# Autodesk Inventor assembly: printer
(part 3 of 3)
- [Mate]: 608RS:5 ↔ CSN 02 1702 B B 8,4:13
- [Mate]: 608RS:5 ↔ CSN 02 1702 B B 8,4:13
- [Mate]: 608RS:6 ↔ rope_pulley:8
- [Mate]: 608RS:6 ↔ rope_pulley:8
- [Mate]: rope_pulley:7 ↔ rope_pulley:8
- [Mate]: rope_pulley:7 ↔ rope_pulley:8
- [Mate]: 608RS:6 ↔ rope_pulley:7
- [Mate]: CSN 02 1702 B B 8,4:15 ↔ CSN 02 1702 B B 8,4:16
- [Mate]: CSN 02 1702 B B 8,4:15 ↔ CSN 02 1702 B B 8,4:16
- [Mate]: CSN 02 1702 B B 8,4:17 ↔ CSN 02 1702 B B 8,4:18
- [Mate]: CSN 02 1702 B B 8,4:17 ↔ CSN 02 1702 B B 8,4:18
- [Mate]: 608RS:6 ↔ CSN 02 1702 B B 8,4:15
- [Mate]: 608RS:6 ↔ CSN 02 1702 B B 8,4:15
- [Mate]: 608RS:6 ↔ CSN 02 1702 B B 8,4:17
- [Mate]: 608RS:6 ↔ CSN 02 1702 B B 8,4:17
- [Mate]: 608RS:7 ↔ rope_pulley:10
- [Mate]: 608RS:7 ↔ rope_pulley:10
- [Mate]: rope_pulley:9 ↔ rope_pulley:10
- [Mate]: rope_pulley:9 ↔ rope_pulley:10
- [Mate]: 608RS:7 ↔ rope_pulley:9
- [Mate]: CSN 02 1702 B B 8,4:19 ↔ CSN 02 1702 B B 8,4:20
- [Mate]: CSN 02 1702 B B 8,4:19 ↔ CSN 02 1702 B B 8,4:20
- [Mate]: CSN 02 1702 B B 8,4:21 ↔ CSN 02 1702 B B 8,4:22
- [Mate]: CSN 02 1702 B B 8,4:21 ↔ CSN 02 1702 B B 8,4:22
- [Mate]: 608RS:7 ↔ CSN 02 1702 B B 8,4:19
- [Mate]: 608RS:7 ↔ CSN 02 1702 B B 8,4:19
- [Mate]: 608RS:7 ↔ CSN 02 1702 B B 8,4:21
- [Mate]: 608RS:7 ↔ CSN 02 1702 B B 8,4:21
- Mate:607: rope_mount_b:1 ↔ CSN 02 1702 B B 8,4:14
- Mate:608: rope_mount_b:1 ↔ CSN 02 1702 B B 8,4:14
- Mate:609: rope_mount_b:1 ↔ CSN 02 1702 B B 8,4:18
- Mate:610: rope_mount_b:1 ↔ CSN 02 1702 B B 8,4:18
- Mate:611: rope_mount_b:2 ↔ CSN 02 1702 B B 8,4:22
- Mate:612: rope_mount_b:2 ↔ CSN 02 1702 B B 8,4:22
- Mate:613: rope_mount_b:2 ↔ CSN 02 1702 B B 8,4:10
- Mate:614: rope_mount_b:2 ↔ CSN 02 1702 B B 8,4:10
- Mate:615: rope_mount_b:2 ↔ CSN 02 1702 B B 8,4:30
- Mate:616: rope_mount_b:2 ↔ CSN 02 1702 B B 8,4:30
- Mate:617: rope_mount_b:2 ↔ CSN 02 1702 B B 8,4:29
- Mate:618: rope_mount_b:2 ↔ CSN 02 1702 B B 8,4:29
- Mate:619: rope_mount_a:1 ↔ CSN 02 1702 B B 8,4:28
- Mate:620: rope_mount_a:1 ↔ CSN 02 1702 B B 8,4:27
- Mate:621: rope_mount_b:1 ↔ CSN 02 1702 B B 8,4:26
- Mate:622: rope_mount_b:1 ↔ CSN 02 1702 B B 8,4:26
- Mate:623: rope_mount_b:1 ↔ CSN 02 1702 B B 8,4:25
- Mate:624: rope_mount_b:1 ↔ CSN 02 1702 B B 8,4:25
- Mate:625: rope_mount_a:2 ↔ CSN 02 1702 B B 8,4:24
- Mate:626: rope_mount_a:2 ↔ CSN 02 1702 B B 8,4:23
- Insert:133: CSN 02 1702 B B 8,4:30 ↔ ISO 4762 M8 x 40:5
- Insert:134: CSN 02 1702 B B 8,4:29 ↔ ISO 4762 M8 x 40:4
- Insert:135: CSN 02 1702 B B 8,4:26 ↔ ISO 4762 M8 x 40:3
- Insert:136: CSN 02 1702 B B 8,4:25 ↔ ISO 4762 M8 x 40:2
- Mate:627: CSN 02 1702 B B 8,4:24 ↔ ISO 4762 M8 x 40:5
- Mate:628: CSN 02 1702 B B 8,4:23 ↔ ISO 4762 M8 x 40:4
- Mate:629: CSN 02 1702 B B 8,4:28 ↔ ISO 4762 M8 x 40:3
- Mate:630: CSN 02 1702 B B 8,4:27 ↔ ISO 4762 M8 x 40:2
- Mate:631: CSN 02 1702 B B 8,4:23 ↔ DIN EN ISO 7040 M8:5
- Mate:632: ISO 4762 M8 x 40:4 ↔ DIN EN ISO 7040 M8:5
- Mate:633: CSN 02 1702 B B 8,4:24 ↔ DIN EN ISO 7040 M8:4
- Mate:634: ISO 4762 M8 x 40:5 ↔ DIN EN ISO 7040 M8:4
- Mate:635: CSN 02 1702 B B 8,4:27 ↔ DIN EN ISO 7040 M8:3
- Mate:636: ISO 4762 M8 x 40:2 ↔ DIN EN ISO 7040 M8:3
- Mate:637: CSN 02 1702 B B 8,4:28 ↔ DIN EN ISO 7040 M8:2
- Mate:638: ISO 4762 M8 x 40:3 ↔ DIN EN ISO 7040 M8:2
- Mate:639: frame:1 ↔ z_axis_top_brace:2
- Mate:640: frame:1 ↔ z_axis_top_brace:2
- Mate:641: z_axis_top:1 ↔ z_axis_top_brace:2
- Mate:642: frame:1 ↔ z_axis_top_brace:1
- Mate:643: z_axis_top:2 ↔ z_axis_top_brace:1
- Mate:644: frame:1 ↔ z_axis_top_brace:1
- Mate:645: z_axis_top:1 ↔ CSN 02 1702 B B 4,3:135
- Mate:646: z_axis_top:1 ↔ CSN 02 1702 B B 4,3:135
- Mate:647: z_axis_top:1 ↔ CSN 02 1702 B B 4,3:137
- Mate:648: z_axis_top:1 ↔ CSN 02 1702 B B 4,3:137
- Mate:649: z_axis_top:2 ↔ CSN 02 1702 B B 4,3:136
- Mate:650: z_axis_top:2 ↔ CSN 02 1702 B B 4,3:136
- Mate:651: z_axis_top:2 ↔ CSN 02 1702 B B 4,3:131
- Mate:652: z_axis_top:2 ↔ CSN 02 1702 B B 4,3:131
- Mate:653: rope_mount_holder:1 ↔ CSN 02 1702 B B 4,3:138
- Mate:654: rope_mount_holder:1 ↔ CSN 02 1702 B B 4,3:138
- Mate:655: rope_mount_holder:1 ↔ CSN 02 1702 B B 4,3:134
- Mate:656: rope_mount_holder:1 ↔ CSN 02 1702 B B 4,3:134
- Mate:657: rope_mount_holder:2 ↔ CSN 02 1702 B B 4,3:133
- Mate:658: rope_mount_holder:2 ↔ CSN 02 1702 B B 4,3:133
- Mate:659: rope_mount_holder:2 ↔ CSN 02 1702 B B 4,3:132
- Mate:660: rope_mount_holder:2 ↔ CSN 02 1702 B B 4,3:132
- Mate:661: frame:1 ↔ CSN 02 1702 B B 4,3:139
- Mate:662: frame:1 ↔ CSN 02 1702 B B 4,3:139
- Mate:663: frame:1 ↔ CSN 02 1702 B B 4,3:146
- Mate:664: frame:1 ↔ CSN 02 1702 B B 4,3:146
- Insert:137: CSN 02 1702 B B 4,3:135 ↔ ISO 4762 M4 x 20:64
- Insert:138: CSN 02 1702 B B 4,3:137 ↔ ISO 4762 M4 x 20:65
- Insert:139: CSN 02 1702 B B 4,3:131 ↔ ISO 4762 M4 x 20:66
- Insert:140: CSN 02 1702 B B 4,3:136 ↔ ISO 4762 M4 x 20:67
- Insert:141: CSN 02 1702 B B 4,3:139 ↔ ISO 4762 M4 x 20:68
- Insert:142: CSN 02 1702 B B 4,3:146 ↔ ISO 4762 M4 x 20:69
- Mate:665: brace_left:1 ↔ CSN 02 1702 B B 4,3:142
- Mate:666: CSN 02 1702 B B 4,3:142 ↔ ISO 4762 M4 x 20:64
- Mate:667: z_axis_top_brace:2 ↔ CSN 02 1702 B B 4,3:145
- Mate:668: CSN 02 1702 B B 4,3:145 ↔ ISO 4762 M4 x 20:68
- Mate:669: frame:1 ↔ CSN 02 1702 B B 4,3:144
- Mate:670: CSN 02 1702 B B 4,3:144 ↔ ISO 4762 M4 x 20:65
- Mate:671: frame:1 ↔ CSN 02 1702 B B 4,3:140
- Mate:672: CSN 02 1702 B B 4,3:140 ↔ ISO 4762 M4 x 20:66
- Mate:673: z_axis_top_brace:1 ↔ CSN 02 1702 B B 4,3:143
- Mate:674: CSN 02 1702 B B 4,3:143 ↔ ISO 4762 M4 x 20:69
- Mate:675: brace_right:1 ↔ CSN 02 1702 B B 4,3:141
- Mate:676: CSN 02 1702 B B 4,3:141 ↔ ISO 4762 M4 x 20:67
- Insert:143: CSN 02 1702 B B 4,3:134 ↔ ISO 4762 M4 x 35:1
- Insert:144: CSN 02 1702 B B 4,3:138 ↔ ISO 4762 M4 x 35:2
- Insert:145: CSN 02 1702 B B 4,3:133 ↔ ISO 4762 M4 x 35:3
- Insert:146: CSN 02 1702 B B 4,3:132 ↔ ISO 4762 M4 x 35:4
- Mate:677: frame:1 ↔ CSN 02 1702 B B 4,3:150
- Mate:678: ISO 4762 M4 x 35:2 ↔ CSN 02 1702 B B 4,3:150
- Mate:679: z_axis_top_brace:2 ↔ CSN 02 1702 B B 4,3:147
- Mate:680: ISO 4762 M4 x 35:1 ↔ CSN 02 1702 B B 4,3:147
- Mate:681: z_axis_top_brace:1 ↔ CSN 02 1702 B B 4,3:148
- Mate:682: ISO 4762 M4 x 35:3 ↔ CSN 02 1702 B B 4,3:148
- Mate:683: frame:1 ↔ CSN 02 1702 B B 4,3:149
- Mate:684: ISO 4762 M4 x 35:4 ↔ CSN 02 1702 B B 4,3:149
- Mate:685: CSN 02 1702 B B 4,3:142 ↔ DIN EN ISO 7040 M4:71
- Mate:686: ISO 4762 M4 x 20:64 ↔ DIN EN ISO 7040 M4:71
- Mate:687: CSN 02 1702 B B 4,3:144 ↔ DIN EN ISO 7040 M4:72
- Mate:688: ISO 4762 M4 x 20:65 ↔ DIN EN ISO 7040 M4:72
- Mate:689: CSN 02 1702 B B 4,3:147 ↔ DIN EN ISO 7040 M4:73
- Mate:690: ISO 4762 M4 x 35:1 ↔ DIN EN ISO 7040 M4:73
- Mate:691: CSN 02 1702 B B 4,3:145 ↔ DIN EN ISO 7040 M4:66
- Mate:692: ISO 4762 M4 x 20:68 ↔ DIN EN ISO 7040 M4:66
- Mate:693: CSN 02 1702 B B 4,3:150 ↔ DIN EN ISO 7040 M4:67
- Mate:694: ISO 4762 M4 x 35:2 ↔ DIN EN ISO 7040 M4:67
- Mate:695: CSN 02 1702 B B 4,3:149 ↔ DIN EN ISO 7040 M4:68
- Mate:696: ISO 4762 M4 x 35:4 ↔ DIN EN ISO 7040 M4:68
- Mate:697: CSN 02 1702 B B 4,3:143 ↔ DIN EN ISO 7040 M4:69
- Mate:698: ISO 4762 M4 x 20:69 ↔ DIN EN ISO 7040 M4:69
- Mate:699: CSN 02 1702 B B 4,3:148 ↔ DIN EN ISO 7040 M4:74
- Mate:700: ISO 4762 M4 x 35:3 ↔ DIN EN ISO 7040 M4:74
- Mate:701: CSN 02 1702 B B 4,3:140 ↔ DIN EN ISO 7040 M4:70
- Mate:702: ISO 4762 M4 x 20:66 ↔ DIN EN ISO 7040 M4:70
- Mate:703: CSN 02 1702 B B 4,3:141 ↔ DIN EN ISO 7040 M4:75
- Mate:704: ISO 4762 M4 x 20:67 ↔ DIN EN ISO 7040 M4:75
- Mate:705: z_axis_top:1 ↔ z_axis_top_cap:1
- Mate:706: z_axis_top:1 ↔ z_axis_top_cap:1
- Mate:707: z_axis_top:1 ↔ z_axis_top_cap:1
- Mate:708: z_axis_top:2 ↔ z_axis_top_cap:2
- Mate:709: z_axis_top:2 ↔ z_axis_top_cap:2
- Mate:710: z_axis_top:2 ↔ z_axis_top_cap:2
- Mate:711: z_axis_top_cap:1 ↔ CSN 02 1702 B B 4,3:154
- Mate:712: z_axis_top_cap:1 ↔ CSN 02 1702 B B 4,3:153
- Mate:713: z_axis_top_cap:1 ↔ CSN 02 1702 B B 4,3:153
- Mate:714: z_axis_top_cap:1 ↔ CSN 02 1702 B B 4,3:154
- Mate:715: z_axis_top_cap:2 ↔ CSN 02 1702 B B 4,3:151
- Mate:716: z_axis_top_cap:2 ↔ CSN 02 1702 B B 4,3:151
- Mate:717: z_axis_top_cap:2 ↔ CSN 02 1702 B B 4,3:152
- Mate:718: z_axis_top_cap:2 ↔ CSN 02 1702 B B 4,3:152
- Insert:147: CSN 02 1702 B B 4,3:154 ↔ ISO 4762 M4 x 20:73
- Insert:148: CSN 02 1702 B B 4,3:153 ↔ ISO 4762 M4 x 20:72
- Insert:149: CSN 02 1702 B B 4,3:151 ↔ ISO 4762 M4 x 20:71
- Insert:150: CSN 02 1702 B B 4,3:152 ↔ ISO 4762 M4 x 20:70
- Mate:719: z_axis_top:1 ↔ CSN 02 1702 B B 4,3:155
- Mate:720: ISO 4762 M4 x 20:72 ↔ CSN 02 1702 B B 4,3:155
- Mate:721: z_axis_top:1 ↔ CSN 02 1702 B B 4,3:156
- Mate:722: ISO 4762 M4 x 20:73 ↔ CSN 02 1702 B B 4,3:156
- Mate:723: z_axis_top:2 ↔ CSN 02 1702 B B 4,3:157
- Mate:724: ISO 4762 M4 x 20:70 ↔ CSN 02 1702 B B 4,3:157
- Mate:725: z_axis_top:2 ↔ CSN 02 1702 B B 4,3:158
- Mate:726: ISO 4762 M4 x 20:71 ↔ CSN 02 1702 B B 4,3:158
- Mate:727: CSN 02 1702 B B 4,3:156 ↔ DIN EN ISO 7040 M4:76
- Mate:728: ISO 4762 M4 x 20:73 ↔ DIN EN ISO 7040 M4:76
- Mate:729: CSN 02 1702 B B 4,3:155 ↔ DIN EN ISO 7040 M4:77
- Mate:730: ISO 4762 M4 x 20:72 ↔ DIN EN ISO 7040 M4:77
- Mate:731: CSN 02 1702 B B 4,3:157 ↔ DIN EN ISO 7040 M4:78
- Mate:732: ISO 4762 M4 x 20:70 ↔ DIN EN ISO 7040 M4:78
- Mate:733: CSN 02 1702 B B 4,3:158 ↔ DIN EN ISO 7040 M4:79
- Mate:734: ISO 4762 M4 x 20:71 ↔ DIN EN ISO 7040 M4:79
- Mate:735: front:1 ↔ y_axis_cap:1
- Mate:736: front:1 ↔ y_axis_cap:2
- Mate:737: back:1 ↔ y_axis_cap:3
- Mate:738: back:1 ↔ y_axis_cap:4
- Mate:739: back:1 ↔ y_axis_cap:4
- Mate:740: back:1 ↔ y_axis_cap:4
- Mate:741: back:1 ↔ y_axis_cap:3
- Mate:742: back:1 ↔ y_axis_cap:3
- Mate:743: front:1 ↔ y_axis_cap:2
- Mate:744: front:1 ↔ y_axis_cap:2
- Mate:745: front:1 ↔ y_axis_cap:1
- Mate:746: front:1 ↔ y_axis_cap:1
- Mate:747: y_axis_cap:1 ↔ CSN 02 1702 B B 4,3:162
- Mate:748: y_axis_cap:1 ↔ CSN 02 1702 B B 4,3:161
- Mate:749: y_axis_cap:2 ↔ CSN 02 1702 B B 4,3:160
- Mate:750: y_axis_cap:2 ↔ CSN 02 1702 B B 4,3:159
- Mate:751: y_axis_cap:3 ↔ CSN 02 1702 B B 4,3:163
- Mate:752: y_axis_cap:3 ↔ CSN 02 1702 B B 4,3:163
- Mate:753: y_axis_cap:3 ↔ CSN 02 1702 B B 4,3:164
- Mate:754: y_axis_cap:3 ↔ CSN 02 1702 B B 4,3:164
- Mate:755: y_axis_cap:4 ↔ CSN 02 1702 B B 4,3:165
- Mate:756: y_axis_cap:4 ↔ CSN 02 1702 B B 4,3:165
- Mate:757: y_axis_cap:4 ↔ CSN 02 1702 B B 4,3:166
- Mate:758: y_axis_cap:4 ↔ CSN 02 1702 B B 4,3:166
- Mate:759: back:1 ↔ CSN 02 1702 B B 4,3:167
- Mate:760: back:1 ↔ CSN 02 1702 B B 4,3:168
- Mate:761: back:1 ↔ CSN 02 1702 B B 4,3:169
- Mate:762: back:1 ↔ CSN 02 1702 B B 4,3:170
- Mate:763: y_axis_cap:1 ↔ CSN 02 1702 B B 4,3:162
- Mate:764: y_axis_cap:1 ↔ CSN 02 1702 B B 4,3:161
- Mate:765: y_axis_cap:2 ↔ CSN 02 1702 B B 4,3:160
- Mate:766: y_axis_cap:2 ↔ CSN 02 1702 B B 4,3:159
- Insert:151: CSN 02 1702 B B 4,3:162 ↔ ISO 4762 M4 x 20:74
- Insert:152: CSN 02 1702 B B 4,3:161 ↔ ISO 4762 M4 x 20:75
- Insert:153: CSN 02 1702 B B 4,3:160 ↔ ISO 4762 M4 x 20:76
- Insert:154: CSN 02 1702 B B 4,3:159 ↔ ISO 4762 M4 x 20:77
- Insert:155: CSN 02 1702 B B 4,3:163 ↔ ISO 4762 M4 x 20:78
- Insert:156: CSN 02 1702 B B 4,3:164 ↔ ISO 4762 M4 x 20:79
- Insert:157: CSN 02 1702 B B 4,3:166 ↔ ISO 4762 M4 x 20:80
- Insert:158: CSN 02 1702 B B 4,3:165 ↔ ISO 4762 M4 x 20:81
- Mate:767: front:1 ↔ CSN 02 1702 B B 4,3:171
- Mate:768: front:1 ↔ CSN 02 1702 B B 4,3:172
- Mate:769: front:1 ↔ CSN 02 1702 B B 4,3:173
- Mate:770: front:1 ↔ CSN 02 1702 B B 4,3:174
- Mate:771: CSN 02 1702 B B 4,3:171 ↔ ISO 4762 M4 x 20:77
- Mate:772: CSN 02 1702 B B 4,3:172 ↔ ISO 4762 M4 x 20:76
- Mate:773: CSN 02 1702 B B 4,3:174 ↔ ISO 4762 M4 x 20:74
- Mate:774: CSN 02 1702 B B 4,3:173 ↔ ISO 4762 M4 x 20:75
- Mate:775: CSN 02 1702 B B 4,3:170 ↔ ISO 4762 M4 x 20:78
- Mate:776: CSN 02 1702 B B 4,3:169 ↔ ISO 4762 M4 x 20:79
- Mate:777: CSN 02 1702 B B 4,3:167 ↔ ISO 4762 M4 x 20:81
- Mate:778: CSN 02 1702 B B 4,3:168 ↔ ISO 4762 M4 x 20:80
- Mate:779: CSN 02 1702 B B 4,3:171 ↔ DIN EN ISO 7040 M4:83
- Mate:780: ISO 4762 M4 x 20:77 ↔ DIN EN ISO 7040 M4:83
- Mate:781: CSN 02 1702 B B 4,3:172 ↔ DIN EN ISO 7040 M4:82
- Mate:782: ISO 4762 M4 x 20:76 ↔ DIN EN ISO 7040 M4:82
- Mate:783: CSN 02 1702 B B 4,3:173 ↔ DIN EN ISO 7040 M4:81
- Mate:784: ISO 4762 M4 x 20:75 ↔ DIN EN ISO 7040 M4:81
- Mate:785: CSN 02 1702 B B 4,3:174 ↔ DIN EN ISO 7040 M4:80
- Mate:786: ISO 4762 M4 x 20:74 ↔ DIN EN ISO 7040 M4:80
- Mate:787: CSN 02 1702 B B 4,3:170 ↔ DIN EN ISO 7040 M4:84
- Mate:788: ISO 4762 M4 x 20:78 ↔ DIN EN ISO 7040 M4:84
- Mate:789: CSN 02 1702 B B 4,3:169 ↔ DIN EN ISO 7040 M4:87
- Mate:790: ISO 4762 M4 x 20:79 ↔ DIN EN ISO 7040 M4:87
- Mate:791: CSN 02 1702 B B 4,3:168 ↔ DIN EN ISO 7040 M4:86
- Mate:792: ISO 4762 M4 x 20:80 ↔ DIN EN ISO 7040 M4:86
- Mate:793: CSN 02 1702 B B 4,3:167 ↔ DIN EN ISO 7040 M4:85
- Mate:794: ISO 4762 M4 x 20:81 ↔ DIN EN ISO 7040 M4:85
- Mate:795: brace_right:1 ↔ IEC inlet:1
- Mate:796: brace_right:1 ↔ IEC inlet:1
- Mate:797: brace_right:1 ↔ IEC inlet:1
- Insert:159: IEC inlet:1 ↔ Cross Recessed Flat Countersunk Head Tapping Screw - Type AB - Type IA - Metric 2,9 x 1 x 8:1
- Insert:160: IEC inlet:1 ↔ Cross Recessed Flat Countersunk Head Tapping Screw - Type AB - Type IA - Metric 2,9 x 1 x 8:2
## Named parameters: d524_d163 = 0 mm, d525_d164 = 0 deg, d526_d165 = 36 deg, d527_d166 = 0 deg, d83_d80 = 0 deg, d84_d81 = 36 deg, d85_d82 = 0 deg, d86_d76 = 0 deg, d87_d77 = 36 deg, d88_d78 = 0 deg, d89_d79 = 0 mm, d90_d75 = 0 mm, d536_d91 = 0 mm, d537_d92 = 0 deg, d538_d93 = 36 deg, d539_d94 = 0 deg, d95_d80 = 0 deg, d96_d81 = 36 deg, d97_d82 = 0 deg, d98_d83_d80 = 0 deg, d99_d84_d81 = 36 deg, d100_d85_d82 = 0 deg, d101_d86_d76 = 0 deg, d102_d87_d77 = 36 deg, d103_d88_d78 = 0 deg, d104_d89_d79 = 0 mm, d105_d90_d75 = 0 mm, d106_d91 = 0 mm, d107_d92 = 0 deg, d108_d93 = 36 deg, d109_d94 = 0 deg, d110_d76 = 0 deg, d111_d77 = 36 deg, d112_d78 = 0 deg, d113_d79 = 0 mm, d114_d75 = 0 mm, d560_d115 = 0 mm, d561_d116 = 0 deg, d562_d117 = 36 deg, d563_d118 = 0 deg, d119_d115 = 0 mm, d120_d116 = 0 deg, d121_d117 = 36 deg, d122_d118 = 0 deg, d123_d80 = 0 deg, d124_d81 = 36 deg, d125_d82 = 0 deg, d126_d83_d80 = 0 deg, d127_d84_d81 = 36 deg, d128_d85_d82 = 0 deg, d129_d86_d76 = 0 deg, d130_d87_d77 = 36 deg, d131_d88_d78 = 0 deg, d132_d89_d79 = 0 mm, d133_d90_d75 = 0 mm, d134_d91 = 0 mm, d135_d92 = 0 deg, d136_d93 = 36 deg, d137_d94 = 0 deg, d153_d110_d76 = 0 deg, d154_d111_d77 = 36 deg, d155_d112_d78 = 0 deg, d157_d114_d75 = 0 mm, d158_d76 = 0 deg, d159_d77 = 36 deg, d160_d78 = 0 deg, d161_d79 = 0 mm, d162_d75 = 0 mm, d608_d75 = 0 mm, d609_d76 = 0 deg, d610_d77 = 36 deg, d611_d78 = 0 deg, d612_d79 = 0 mm, d613_d80 = 0 deg, d614_d81 = 36 deg, d615_d82 = 0 deg, d632_d163 = 0 mm, d633_d164 = 0 deg, d634_d165 = 36 deg, d635_d166 = 0 deg, d636_d83_d80 = 0 deg, d637_d84_d81 = 36 deg, d638_d85_d82 = 0 deg, d639_d86_d76 = 0 deg, d640_d87_d77 = 36 deg, d641_d88_d78 = 0 deg, d642_d89_d79 = 0 mm, d643_d90_d75 = 0 mm, d644_d91 = 0 mm, d645_d92 = 0 deg, d646_d93 = 36 deg, d647_d94 = 0 deg, d648_d95_d80 = 0 deg, d649_d96_d81 = 36 deg, d650_d97_d82 = 0 deg, d651_d98_d83_d80 = 0 deg, d652_d99_d84_d81 = 36 deg, d653_d100_d85_d82 = 0 deg, d654_d101_d86_d76 = 0 deg, d655_d102_d87_d77 = 36 deg, d656_d103_d88_d78 = 0 deg, d657_d104_d89_d79 = 0 mm, d658_d105_d90_d75 = 0 mm, d659_d106_d91 = 0 mm, d660_d107_d92 = 0 deg, d661_d108_d93 = 36 deg, d662_d109_d94 = 0 deg, d663_d110_d76 = 0 deg, d664_d111_d77 = 36 deg, d665_d112_d78 = 0 deg, d666_d113_d79 = 0 mm, d667_d114_d75 = 0 mm, d668_d115 = 0 mm, d669_d116 = 0 deg, d670_d117 = 36 deg, d671_d118 = 0 deg, d672_d119_d115 = 0 mm, d673_d120_d116 = 0 deg, d674_d121_d117 = 36 deg, d675_d122_d118 = 0 deg, d676_d123_d80 = 0 deg, d677_d124_d81 = 36 deg, d678_d125_d82 = 0 deg, d679_d126_d83_d80 = 0 deg, d680_d127_d84_d81 = 36 deg, d681_d128_d85_d82 = 0 deg, d682_d129_d86_d76 = 0 deg, d683_d130_d87_d77 = 36 deg, d684_d131_d88_d78 = 0 deg, d685_d132_d89_d79 = 0 mm, d686_d133_d90_d75 = 0 mm, d687_d134_d91 = 0 mm, d688_d135_d92 = 0 deg, d689_d136_d93 = 36 deg, d690_d137_d94 = 0 deg, d138_d95_d80 = 0 deg, d139_d96_d81 = 36 deg, d140_d97_d82 = 0 deg, d141_d98_d83_d80 = 0 deg, d142_d99_d84_d81 = 36 deg, d143_d100_d85_d82 = 0 deg, d144_d101_d86_d76 = 0 deg, d145_d102_d87_d77 = 36 deg, d146_d103_d88_d78 = 0 deg, d147_d104_d89_d79 = 0 mm, d148_d105_d90_d75 = 0 mm, d149_d106_d91 = 0 mm, d150_d107_d92 = 0 deg, d151_d108_d93 = 36 deg, d152_d109_d94 = 0 deg, d706_d153_d110_d76 = 0 deg, d707_d154_d111_d77 = 36 deg, d708_d155_d112_d78 = 0 deg, d156_d113_d79 = 0 mm, d710_d157_d114_d75 = 0 mm, d711_d158_d76 = 0 deg, d712_d159_d77 = 36 deg, d713_d160_d78 = 0 deg, d714_d161_d79 = 0 mm, d715_d162_d75 = 0 mm, d720_d79 = 0 mm, d721_d80 = 0 deg, d722_d81 = 36 deg, d723_d82 = 0 deg, d957_d949 = 0 mm, d958_d950 = 0 mm, d959_d951 = 0 mm, d960_d952 = 0 mm, d961_d953 = 0 mm, d962_d954 = 0 mm, d963_d955 = 0 mm, d964_d956 = 0 mm, d965_d937 = 0 mm, d966_d943 = 0 mm, d967_d944 = 0 mm, d968_d945 = 0 mm, d969_d946 = 0 mm, d970_d949 = 0 mm, d971_d950 = 0 mm, d972_d951 = 0 mm, d973_d952 = 0 mm, d974_d953 = 0 mm, d975_d954 = 0 mm, d976_d955 = 0 mm, d977_d956 = 0 mm, d978_d937 = 0 mm, d979_d943 = 0 mm, d980_d944 = 0 mm, d981_d945 = 0 mm, d982_d946 = 0 mm, d983_d949 = 0 mm, d984_d950 = 0 mm, d985_d951 = 0 mm, d986_d952 = 0 mm, d987_d953 = 0 mm, d988_d954 = 0 mm, d989_d955 = 0 mm, d990_d956 = 0 mm, d991_d937 = 0 mm, d992_d943 = 0 mm, d993_d944 = 0 mm, d994_d945 = 0 mm, d995_d946 = 0 mm
